# Autodesk Inventor assembly: motor_acople
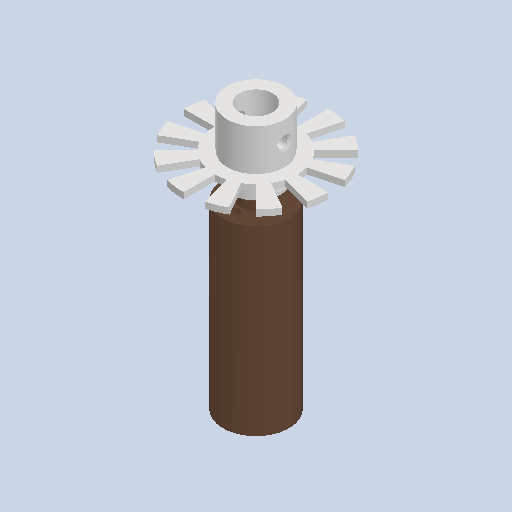
[picture p0: Inventor's stored thumbnail of the model, 512x512]
Saved by Autodesk Inventor 2024.2 (Build 282272000, 272)
## iProperties
Created: 2022-12-05
Part Number: motor_acople
Document SubType Name: Assembly
Designer: sergi
Author: sergi
## Documents named in this file (4)
- C:\Users\sergi\OneDrive\Escritorio\Projects\Automatic Feeder\ComederoV4\Inventor\motor_acople.iam
- C:\Users\sergi\OneDrive\Escritorio\Projects\Automatic Feeder\ComederoV4\Inventor\motor2.ipt
- C:\Users\sergi\OneDrive\Escritorio\Projects\Automatic Feeder\ComederoV4\Inventor\Acople2.ipt
- C:\Users\sergi\OneDrive\Escritorio\Projects\Automatic Feeder\ComederoV4\Inventor\Encoder2.ipt
## Components (3 placed, 3 different names)
1. motor2:1 — Coincidencia:3, Coincidencia:4
2. Acople2:1 — Coincidencia:1, Coincidencia:2, Coincidencia:3, Coincidencia:4
3. Encoder2:1 — Coincidencia:1, Coincidencia:2
## Relationships (4: Mate 4)
- Coincidencia:1 [Mate]: Acople2:1 ↔ Encoder2:1
- Coincidencia:2 [Mate]: Acople2:1 ↔ Encoder2:1
- Coincidencia:3 [Mate]: motor2:1 ↔ Acople2:1
- Coincidencia:4 [Mate] (2 mm): motor2:1 ↔ Acople2:1
